# Autodesk Inventor assembly: M2-M-脚クランク原動節v2
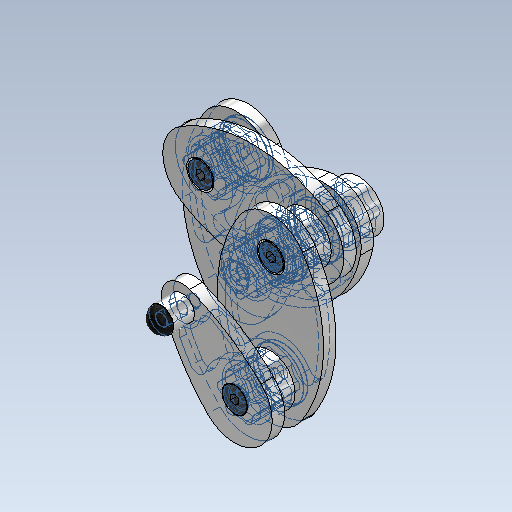
[picture p0: Inventor's stored thumbnail of the model, 512x512]
Saved by Autodesk Inventor 2020 (Build 240168000, 168)
## iProperties
Created: 2021-02-21
Part Number: M2-M-脚クランク原動節v2
Document SubType Name: Assembly
Designer: AA19065
Mass: 32.3437 g
Surface Area: 166.98 cm^2
Volume: 10.8444 cm^3
Density: 2.98252 g/cm^3
Author: AA19065
## Documents named in this file (10)
- C:\Users\happy\OneDrive\ドキュメント\賢一ファイル\SRDC\試作10-2\アセンブリ\M2-M-脚クランク原動節v2.iam
- C:\Users\happy\OneDrive\ドキュメント\賢一ファイル\SRDC\試作10-2\脚クランク\原動節v2\M2-M-原動節0v2.ipt
- C:\Users\happy\OneDrive\ドキュメント\賢一ファイル\SRDC\試作10-2\脚クランク\原動節v2\M2-M-原動節1-3v2.ipt
- C:\Users\happy\OneDrive\ドキュメント\賢一ファイル\SRDC\試作10-2\脚クランク\原動節v2\M2-M-原動節4v2.ipt
- C:\Users\happy\OneDrive\ドキュメント\賢一ファイル\SRDC\試作10-2\脚クランク\原動節v2\M2-M-原動節接続部v2外.ipt
- C:\Users\happy\OneDrive\ドキュメント\賢一ファイル\SRDC\試作10-2\脚クランク\原動節v2\M2-M-原動節接続部v2内-1.ipt
- C:\Users\happy\OneDrive\ドキュメント\賢一ファイル\SRDC\試作10-2\脚クランク\原動節v2\M2-M-原動節接続部v2内-2.ipt
- C:\Users\happy\OneDrive\ドキュメント\賢一ファイル\SRDC\試作10-2\ねじ\M2-M-m3皿ネジ10 (1).ipt
- C:\Users\happy\OneDrive\ドキュメント\賢一ファイル\SRDC\試作10-2\スペーサ\M2-M-5mm.ipt
- C:\Users\happy\OneDrive\ドキュメント\賢一ファイル\SRDC\試作10-2\ねじ\M2-M-M3ボタンボルト8.ipt
## Components (25 placed, 9 different names)
1. M2-M-原動節0v2:1 — 挿入:36, 挿入:37, 挿入:13, 挿入:26, 挿入:58, 挿入:59, 挿入:60
2. M2-M-原動節1-3v2:1 — 挿入:19, 挿入:25, 挿入:38, 挿入:39, 挿入:30, 挿入:31, 挿入:53
3. M2-M-原動節4v2:1 — 挿入:34, 挿入:35, 挿入:55, 挿入:56
4. M2-M-原動節接続部v2外:1 — 挿入:36, 挿入:37
5. M2-M-原動節接続部v2内-1:1 — 挿入:19, 挿入:25, 挿入:48, 挿入:49
6. M2-M-原動節接続部v2内-2:1 — 挿入:34, 挿入:35, 挿入:50, 挿入:51
7. M2-M-原動節1-3v2:2 — 挿入:17, 挿入:27, 挿入:28, 挿入:29, 挿入:42, 挿入:43, 挿入:54
8. M2-M-原動節1-3v2:3 — 挿入:40, 挿入:41, 挿入:22, 挿入:24, 挿入:32, 挿入:33, 挿入:52
9. M2-M-原動節接続部v2外:2 — 挿入:38, 挿入:39
10. M2-M-原動節接続部v2内-1:2 — 挿入:17, 挿入:27, 挿入:46, 挿入:47
11. M2-M-原動節接続部v2内-2:2 — 挿入:28, 挿入:29, 挿入:44, 挿入:45
12. M2-M-原動節接続部v2外:3 — 挿入:40, 挿入:41
13. M2-M-原動節接続部v2内-1:3 — 挿入:13, 挿入:26, 挿入:44, 挿入:45
14. M2-M-原動節接続部v2内-2:3 — 挿入:30, 挿入:31, 挿入:46, 挿入:47
15. M2-M-原動節接続部v2外:4 — 挿入:42, 挿入:43
16. M2-M-原動節接続部v2内-1:4 — 挿入:22, 挿入:24, 挿入:50, 挿入:51
17. M2-M-原動節接続部v2内-2:4 — 挿入:32, 挿入:33, 挿入:48, 挿入:49
18. M2-M-m3皿ネジ10 (1):1 — 挿入:55
19. M2-M-m3皿ネジ10 (1):2 — 挿入:54
20. M2-M-m3皿ネジ10 (1):3 — 挿入:53
21. M2-M-m3皿ネジ10 (1):4 — 挿入:52
22. M2-M-5mm:1 — 挿入:56, 挿入:57
23. M2-M-M3ボタンボルト8:1 — 挿入:57
24. M2-M-原動節接続部v2内-2:5 — 挿入:58, 挿入:59, メイト:1
25. M2-M-原動節接続部v2外:5 — 挿入:60, メイト:1
## Relationships (42: Insert 41, Mate 1)
- 挿入:36 [Insert]: M2-M-原動節0v2:1 ↔ M2-M-原動節接続部v2外:1
- 挿入:37 [Insert]: M2-M-原動節0v2:1 ↔ M2-M-原動節接続部v2外:1
- 挿入:19 [Insert]: M2-M-原動節1-3v2:1 ↔ M2-M-原動節接続部v2内-1:1
- 挿入:25 [Insert]: M2-M-原動節1-3v2:1 ↔ M2-M-原動節接続部v2内-1:1
- 挿入:34 [Insert]: M2-M-原動節4v2:1 ↔ M2-M-原動節接続部v2内-2:1
- 挿入:35 [Insert]: M2-M-原動節4v2:1 ↔ M2-M-原動節接続部v2内-2:1
- 挿入:38 [Insert]: M2-M-原動節1-3v2:1 ↔ M2-M-原動節接続部v2外:2
- 挿入:39 [Insert]: M2-M-原動節1-3v2:1 ↔ M2-M-原動節接続部v2外:2
- 挿入:17 [Insert]: M2-M-原動節1-3v2:2 ↔ M2-M-原動節接続部v2内-1:2
- 挿入:27 [Insert]: M2-M-原動節1-3v2:2 ↔ M2-M-原動節接続部v2内-1:2
- 挿入:28 [Insert]: M2-M-原動節1-3v2:2 ↔ M2-M-原動節接続部v2内-2:2
- 挿入:29 [Insert]: M2-M-原動節1-3v2:2 ↔ M2-M-原動節接続部v2内-2:2
- 挿入:40 [Insert]: M2-M-原動節1-3v2:3 ↔ M2-M-原動節接続部v2外:3
- 挿入:41 [Insert]: M2-M-原動節1-3v2:3 ↔ M2-M-原動節接続部v2外:3
- 挿入:13 [Insert]: M2-M-原動節0v2:1 ↔ M2-M-原動節接続部v2内-1:3
- 挿入:26 [Insert]: M2-M-原動節0v2:1 ↔ M2-M-原動節接続部v2内-1:3
- 挿入:44 [Insert] (0.5 mm): M2-M-原動節接続部v2内-2:2 ↔ M2-M-原動節接続部v2内-1:3
- 挿入:45 [Insert] (0.5 mm): M2-M-原動節接続部v2内-2:2 ↔ M2-M-原動節接続部v2内-1:3
- 挿入:30 [Insert]: M2-M-原動節1-3v2:1 ↔ M2-M-原動節接続部v2内-2:3
- 挿入:31 [Insert]: M2-M-原動節1-3v2:1 ↔ M2-M-原動節接続部v2内-2:3
- 挿入:46 [Insert] (0.5 mm): M2-M-原動節接続部v2内-1:2 ↔ M2-M-原動節接続部v2内-2:3
- 挿入:47 [Insert] (0.5 mm): M2-M-原動節接続部v2内-1:2 ↔ M2-M-原動節接続部v2内-2:3
- 挿入:42 [Insert]: M2-M-原動節1-3v2:2 ↔ M2-M-原動節接続部v2外:4
- 挿入:43 [Insert]: M2-M-原動節1-3v2:2 ↔ M2-M-原動節接続部v2外:4
- 挿入:22 [Insert]: M2-M-原動節1-3v2:3 ↔ M2-M-原動節接続部v2内-1:4
- 挿入:24 [Insert]: M2-M-原動節1-3v2:3 ↔ M2-M-原動節接続部v2内-1:4
- 挿入:50 [Insert] (0.5 mm): M2-M-原動節接続部v2内-2:1 ↔ M2-M-原動節接続部v2内-1:4
- 挿入:51 [Insert] (0.5 mm): M2-M-原動節接続部v2内-2:1 ↔ M2-M-原動節接続部v2内-1:4
- 挿入:32 [Insert]: M2-M-原動節1-3v2:3 ↔ M2-M-原動節接続部v2内-2:4
- 挿入:33 [Insert]: M2-M-原動節1-3v2:3 ↔ M2-M-原動節接続部v2内-2:4
- 挿入:48 [Insert] (0.5 mm): M2-M-原動節接続部v2内-1:1 ↔ M2-M-原動節接続部v2内-2:4
- 挿入:49 [Insert] (0.5 mm): M2-M-原動節接続部v2内-1:1 ↔ M2-M-原動節接続部v2内-2:4
- 挿入:55 [Insert]: M2-M-原動節4v2:1 ↔ M2-M-m3皿ネジ10 (1):1
- 挿入:54 [Insert]: M2-M-原動節1-3v2:2 ↔ M2-M-m3皿ネジ10 (1):2
- 挿入:53 [Insert]: M2-M-原動節1-3v2:1 ↔ M2-M-m3皿ネジ10 (1):3
- 挿入:52 [Insert]: M2-M-原動節1-3v2:3 ↔ M2-M-m3皿ネジ10 (1):4
- 挿入:56 [Insert]: M2-M-原動節4v2:1 ↔ M2-M-5mm:1
- 挿入:57 [Insert]: M2-M-5mm:1 ↔ M2-M-M3ボタンボルト8:1
- 挿入:58 [Insert]: M2-M-原動節0v2:1 ↔ M2-M-原動節接続部v2内-2:5
- 挿入:59 [Insert]: M2-M-原動節0v2:1 ↔ M2-M-原動節接続部v2内-2:5
- 挿入:60 [Insert]: M2-M-原動節0v2:1 ↔ M2-M-原動節接続部v2外:5
- メイト:1 [Mate]: M2-M-原動節接続部v2内-2:5 ↔ M2-M-原動節接続部v2外:5
